# Autodesk Inventor assembly: AX-01 CoreXY
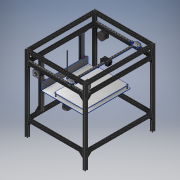
[picture p0: Inventor's stored thumbnail of the model, 180x180]
Saved by Autodesk Inventor 2017.3 (Build 213256000, 256)
## iProperties
Created: 2018-10-06
Part Number: AX-01 CoreXY
Document SubType Name: Assembly
Designer: Ax
Author: Ax
## Documents named in this file (36)
- C:\Users\Ax\Documents\Inventor\AX-01\AX-01 CoreXY.iam
- C:\Users\Ax\Documents\Inventor\Content Center Files\R2017\en-US\V-Slot 20 x 20\20-20-V-slot 20 mm x 20 mm-Aluminum 6061-470.ipt
- C:\Users\Ax\Documents\Inventor\Content Center Files\R2017\en-US\V-Slot 20 x 20\20-20-V-slot 20 mm x 20 mm-Aluminum 6061-550.ipt
- C:\Users\Ax\Documents\Inventor\Content Center Files\R2017\en-US\V-Slot 20 x 20\20-20-V-slot 20 mm x 20 mm-Aluminum 6061-400.ipt
- C:\Users\Ax\Documents\Inventor\Content Center Files\R2017\en-US\V-Slot 20 x 20\20-20-V-slot 20 mm x 20 mm-Aluminum 6061-340.ipt
- C:\Users\Ax\Documents\Inventor\AX-01\Bed Base.ipt
- C:\Users\Ax\Documents\Inventor\Drakon\Library\mgn12-sliding-block-linear-guide-1.snapshot.2\MGN12 Rail 300mm.ipt
- C:\Users\Ax\Documents\Inventor\Drakon\Library\mgn12-sliding-block-linear-guide-1.snapshot.2\MGN12H Block.iam
- C:\Users\Ax\Documents\Inventor\Drakon\Library\mgn12-sliding-block-linear-guide-1.snapshot.2\MGN12 Rail 300mm_MIR.ipt
- C:\Users\Ax\Documents\Inventor\Drakon\Library\mgn12-sliding-block-linear-guide-1.snapshot.2\MGN12H Block_MIR.iam
- C:\Users\Ax\Documents\Inventor\Drakon\Library\MGN9 Rail 400mm.ipt
- C:\Users\Ax\Documents\Inventor\Drakon\Library\MGN9C Block.ipt
- C:\Users\Ax\Documents\Inventor\Drakon\Library\MGN9 Rail 400mm_MIR.ipt
- C:\Users\Ax\Documents\Inventor\Drakon\Library\MGN9C Block_MIR.ipt
- C:\Users\Ax\Documents\Inventor\AX-01\Bed Plate.ipt
- C:\Users\Ax\Documents\Inventor\Drakon\Library\20mm Nylon Stand Off.ipt
- C:\Users\Ax\Documents\Inventor\AX-01\Internal Base Cladding.ipt
- C:\Users\Ax\Documents\Inventor\Drakon\Library\Nema 17 Motor.ipt
- C:\Users\Ax\Documents\Inventor\AX-01\300mmx8mm Lead Screw.ipt
- C:\Users\Ax\Documents\Inventor\Drakon\Library\Rigid_Coupler_5mm_8mm.iam
- C:\Users\Ax\Documents\Inventor\AX-01\TR8 Leadscrew Nut.ipt
- C:\Users\Ax\Documents\Inventor\AX-01\XY_Plate.ipt
- C:\Users\Ax\Documents\Inventor\AX-01\MGN-9 Rail 470mm.ipt
- C:\Users\Ax\Documents\Inventor\Content Center Files\R2017\en-US\ISO 4762(2)\ISO 4762 - M3 x 6ISO.ipt
- C:\Users\Ax\Documents\Inventor\AX-01\Back Cladding.ipt
- C:\Users\Ax\Documents\Inventor\AX-01\Side Cladding.ipt
- C:\Users\Ax\Documents\Inventor\AX-01\Front Cladding.ipt
- C:\Users\Ax\Documents\Inventor\AX-01\Top Cladding.ipt
- C:\Users\Ax\Documents\Inventor\AX-01\Corner Bracket.ipt
- C:\Users\Ax\Documents\Inventor\AX-01\Idler Pulley.iam
- C:\Users\Ax\Documents\Inventor\AX-01\XY_Carriage.ipt
- C:\Users\Ax\Documents\Inventor\AX-01\Idler Left.ipt
- C:\Users\Ax\Documents\Inventor\AX-01\XY_Tensioner.ipt
- C:\Users\Ax\Documents\Inventor\AX-01\XY_Metal_Slug.ipt
- C:\Users\Ax\Documents\Inventor\AX-01\M3 Conical Washer.ipt
- C:\Users\Ax\Documents\Inventor\AX-01\6mm XY Packer Block.ipt
## Components (114 placed, 35 different names)
1. Bed Base:1 — Mate:24, Mate:38, Mate:39, Flush:46, Mate:40, Mate:41, Mate:42, Mate:43, Mate:44, Mate:45, Mate:46, Mate:47, Mate:48, Mate:49, Mate:61, Mate:62, Mate:63
2. Bed Plate:1 — Mate:38, Mate:39, Flush:46
3. 20mm Nylon Stand Off:1 — Mate:46, Mate:47
4. 20mm Nylon Stand Off:2 — Mate:44, Mate:45
5. 20mm Nylon Stand Off:3 — Mate:40, Mate:41
6. 20mm Nylon Stand Off:4 — Mate:42, Mate:43
7. 300mmx8mm Lead Screw:1 — Mate:57, Mate:58
8. Rigid_Coupler_5mm_8mm:1 [sub-assembly] — Mate:57, Mate:58, Mate:59, Mate:60
9. TR8 Leadscrew Nut:1 — Mate:61, Mate:62, Mate:63
10. XY_Plate:1 — Mate:65, Mate:66, Mate:67, Mate:68, Mate:69, Mate:70, Insert:1, Insert:2, Insert:3, Insert:4, Mate:130, Mate:131, Rotational:4, Rotational:6, Rotational:7, Insert:6, Insert:7, Insert:8, Insert:9, Mate:172
11. Idler Pulley:2 [sub-assembly] — Mate:130, Mate:131
12. Idler Pulley:6 [sub-assembly] — Rotational:6
13. Idler Pulley:7 [sub-assembly] — Rotational:4
14. Idler Pulley:8 [sub-assembly] — Rotational:7
15. XY_Carriage:1 — Mate:151, Mate:152, Mate:153, Mate:154, Mate:155, Mate:156, Mate:157, Mate:158, Mate:159, Mate:160, Mate:161, Mate:162, Mate:163, Mate:164, Mate:165, Mate:166, Mate:167, Mate:168, Mate:169
16. Idler Left:1 — Mate:149, Mate:150, Flush:85
17. XY_Tensioner:1 — Mate:154, Mate:155, Mate:156
18. XY_Tensioner:2 — Mate:157, Mate:158, Mate:159
19. XY_Metal_Slug:1 — Mate:160, Mate:161
20. M3 Conical Washer:1 — Mate:163, Mate:169
21. M3 Conical Washer:2 — Mate:164, Mate:168
22. M3 Conical Washer:3 — Mate:162, Mate:167
23. M3 Conical Washer:4 — Mate:165, Mate:166
24. 6mm XY Packer Block:1 — Mate:170, Flush:86, Flush:87
25. 6mm XY Packer Block:2 — Mate:171, Flush:88, Flush:89, Mate:172
26. V-Slot 20 x 20 20-20-V-slot 20 mm x 20 mm-Aluminum 6061-340:2 — Flush:33, Flush:34, Mate:25, Mate:27, Mate:33, Flush:41, Flush:72, Mate:104, Flush:73, Mate:107, Flush:74, Mate:109
27. V-Slot 20 x 20 20-20-V-slot 20 mm x 20 mm-Aluminum 6061-340:1 — Mate:21, Mate:22, Flush:28, Flush:29, Mate:32, Flush:40, Mate:101, Flush:71, Mate:102, Flush:75, Mate:110, Flush:76, Mate:112
28. V-Slot 20 x 20 20-20-V-slot 20 mm x 20 mm-Aluminum 6061-550:1 — Mate:1, Flush:1, Flush:2, Mate:3, Flush:5, Flush:6, Mate:19, Flush:25, Flush:26, Flush:67, Mate:94, Flush:68, Mate:97, Flush:78, Mate:116, Flush:79, Mate:118
29. V-Slot 20 x 20 20-20-V-slot 20 mm x 20 mm-Aluminum 6061-550:2 — Mate:2, Flush:3, Flush:4, Mate:4, Flush:7, Mate:37, Mate:73, Mate:88, Flush:66, Mate:92, Flush:77, Mate:114, Flush:84, Mate:128
30. V-Slot 20 x 20 20-20-V-slot 20 mm x 20 mm-Aluminum 6061-470:1 — Mate:1, Flush:1, Flush:2, Mate:2, Flush:3, Flush:4, Mate:33, Flush:41, Mate:93, Mate:95, Flush:70, Mate:100, Mate:103, Mate:105, Mate:106
31. V-Slot 20 x 20 20-20-V-slot 20 mm x 20 mm-Aluminum 6061-470:2 — Mate:4, Flush:7, Mate:30, Mate:32, Flush:40, Mate:74, Mate:108, Mate:111, Mate:113, Mate:115, Mate:117
32. V-Slot 20 x 20 20-20-V-slot 20 mm x 20 mm-Aluminum 6061-470:3 — Mate:3, Flush:5, Flush:6, Mate:30
33. V-Slot 20 x 20 20-20-V-slot 20 mm x 20 mm-Aluminum 6061-550:3 — Flush:13, Mate:15, Mate:16, Mate:17, Flush:20, Flush:21, Flush:22, Flush:23, Flush:24, Mate:27, Flush:36, Mate:35, Flush:52, Flush:62, Mate:85, Flush:69, Mate:98, Flush:80, Mate:120, Flush:81, Mate:122, Mate:149
34. V-Slot 20 x 20 20-20-V-slot 20 mm x 20 mm-Aluminum 6061-550:4 — Mate:11, Flush:15, Flush:16, Mate:12, Flush:17, Mate:14, Flush:18, Flush:19, Mate:21, Flush:37, Flush:38, Flush:39, Mate:86, Flush:63, Flush:64, Mate:91, Flush:65, Flush:82, Mate:124, Flush:83, Mate:126
35. V-Slot 20 x 20 20-20-V-slot 20 mm x 20 mm-Aluminum 6061-470:4 — Flush:47, Mate:84, Mate:87
36. V-Slot 20 x 20 20-20-V-slot 20 mm x 20 mm-Aluminum 6061-470:5 — Mate:28, Mate:123, Mate:125, Mate:150, Flush:85
37. V-Slot 20 x 20 20-20-V-slot 20 mm x 20 mm-Aluminum 6061-470:6 — Flush:13, Mate:28, Mate:76
38. V-Slot 20 x 20 20-20-V-slot 20 mm x 20 mm-Aluminum 6061-400:1 — Mate:17, Flush:22, Flush:24, Mate:29, Mate:72, Flush:51, Mate:77
39. V-Slot 20 x 20 20-20-V-slot 20 mm x 20 mm-Aluminum 6061-400:2 — Mate:16, Flush:21, Mate:29, Mate:34, Flush:43, Mate:119, Mate:121
40. V-Slot 20 x 20 20-20-V-slot 20 mm x 20 mm-Aluminum 6061-400:3 — Mate:12, Flush:17, Mate:31, Mate:36, Flush:45, Mate:127, Mate:129
41. V-Slot 20 x 20 20-20-V-slot 20 mm x 20 mm-Aluminum 6061-400:4 — Mate:15, Flush:20, Flush:23, Mate:19, Flush:25, Flush:26, Mate:96, Mate:99
42. V-Slot 20 x 20 20-20-V-slot 20 mm x 20 mm-Aluminum 6061-400:5 — Mate:14, Flush:18, Flush:19, Mate:31, Flush:53
43. V-Slot 20 x 20 20-20-V-slot 20 mm x 20 mm-Aluminum 6061-400:6 — Mate:11, Flush:15, Flush:16, Mate:50, Flush:48, Mate:89, Mate:90
44. Internal Base Cladding:1 — Mate:50, Flush:47, Flush:48, Mate:51, Mate:52, Mate:53
45. Top Cladding:1 — Mate:77, Flush:60, Flush:61
46. Back Cladding:1 — Mate:74, Flush:56, Mate:75, Flush:57
47. Side Cladding:1 — Mate:73, Flush:53, Mate:75, Flush:57, Flush:58, Flush:59, Mate:78, Mate:79, Mate:80
48. Side Cladding:2 — Mate:72, Flush:51, Flush:52, Flush:56, Flush:60, Mate:81, Mate:82, Mate:83
49. Front Cladding:1 — Mate:76, Flush:58, Flush:59, Flush:61
50. MGN9C Block:2 — Slider:5, Mate:151, Mate:152, Mate:153
51. MGN-9 Rail 470mm:1 — Mate:68, Mate:69, Mate:70, Slider:5, Insert:5
52. MGN9C Block_MIR:1 — Slider:4, Mate:66, Mate:67, Mate:171, Flush:88, Flush:89
53. MGN9 Rail 400mm_MIR:1 — Slider:4, Mate:36, Mate:37, Flush:45
54. MGN9C Block:1 — Slider:3, Mate:65, Mate:170, Flush:86, Flush:87
55. MGN9 Rail 400mm:1 — Mate:34, Mate:35, Flush:43, Slider:3
56. MGN12H Block_MIR:1 [sub-assembly] — Mate:26, Slider:2, Mate:48
57. MGN12H Block:1 [sub-assembly] — Mate:23, Slider:1, Mate:24, Mate:49
58. MGN12 Rail 300mm:1 — Mate:22, Flush:28, Flush:29, Mate:23, Slider:1
59. MGN12 Rail 300mm_MIR:1 — Flush:33, Flush:34, Mate:25, Mate:26, Slider:2
60. Nema 17 Motor:2 — Mate:81, Mate:82, Mate:83
61. Nema 17 Motor:3 — Mate:78, Mate:79, Mate:80
62. Nema 17 Motor:1 — Mate:51, Mate:52, Mate:53, Mate:59, Mate:60
63. ISO 4762 M3 x 6:33 — Insert:8
64. ISO 4762 M3 x 6:34 — Insert:9
65. ISO 4762 M3 x 6:35 — Insert:6
66. ISO 4762 M3 x 6:36 — Insert:7
67. ISO 4762 M3 x 6:1 — Insert:3
68. ISO 4762 M3 x 6:2 — Insert:4
69. ISO 4762 M3 x 6:3 — Insert:1
70. ISO 4762 M3 x 6:4 — Insert:2
71. Corner Bracket:1 — Mate:84, Flush:62, Mate:85
72. Corner Bracket:2 — Flush:64, Mate:88, Mate:89
73. Corner Bracket:3 — Mate:86, Flush:63, Mate:87
74. Corner Bracket:4 — Flush:66, Mate:92, Mate:93
75. Corner Bracket:5 — Flush:67, Mate:94, Mate:95
76. Corner Bracket:6 — Mate:90, Mate:91, Flush:65
77. Corner Bracket:7 — Flush:83, Mate:126, Mate:127
78. Corner Bracket:8 — Flush:69, Mate:98, Mate:99
79. Corner Bracket:9 — Flush:68, Mate:96, Mate:97
80. Corner Bracket:10 — Flush:75, Mate:110, Mate:111
81. Corner Bracket:11 — Flush:70, Mate:100, Mate:101
82. Corner Bracket:12 — Flush:76, Mate:112, Mate:113
83. Corner Bracket:13 — Flush:78, Mate:116, Mate:117
84. Corner Bracket:14 — Flush:74, Mate:108, Mate:109
85. Corner Bracket:15 — Flush:72, Mate:104, Mate:105
86. Corner Bracket:16 — Flush:71, Mate:102, Mate:103
87. Corner Bracket:17 — Flush:73, Mate:106, Mate:107
88. Corner Bracket:18 — Flush:77, Mate:114, Mate:115
89. Corner Bracket:19 — Flush:82, Mate:124, Mate:125
90. Corner Bracket:20 — Flush:81, Mate:122, Mate:123
91. Corner Bracket:21 — Flush:79, Mate:118, Mate:119
92. Corner Bracket:22 — Flush:80, Mate:120, Mate:121
93. Corner Bracket:23 — Flush:84, Mate:128, Mate:129
94. ISO 4762 M3 x 6:12 — Insert:5
95. ISO 4762 M3 x 6:13
96. ISO 4762 M3 x 6:14
97. ISO 4762 M3 x 6:15
98. ISO 4762 M3 x 6:16
99. ISO 4762 M3 x 6:17
100. ISO 4762 M3 x 6:18
101. ISO 4762 M3 x 6:19
102. ISO 4762 M3 x 6:20
103. ISO 4762 M3 x 6:21
104. ISO 4762 M3 x 6:22
105. ISO 4762 M3 x 6:23
106. ISO 4762 M3 x 6:24
107. ISO 4762 M3 x 6:25
108. ISO 4762 M3 x 6:26
109. ISO 4762 M3 x 6:27
110. ISO 4762 M3 x 6:28
111. ISO 4762 M3 x 6:29
112. ISO 4762 M3 x 6:30
113. ISO 4762 M3 x 6:31
114. ISO 4762 M3 x 6:32
## Component patterns: (21 elements, first: ISO 4762 M3 x 6:12)
## Relationships (241: Mate 145, Flush 79, Insert 9, TranslationJoint 5, RevoluteJoint 3)
- Mate:1: V-Slot 20 x 20 20-20-V-slot 20 mm x 20 mm-Aluminum 6061-550:1 ↔ V-Slot 20 x 20 20-20-V-slot 20 mm x 20 mm-Aluminum 6061-470:1
- Flush:1 (100 mm): V-Slot 20 x 20 20-20-V-slot 20 mm x 20 mm-Aluminum 6061-550:1 ↔ V-Slot 20 x 20 20-20-V-slot 20 mm x 20 mm-Aluminum 6061-470:1
- Flush:2: V-Slot 20 x 20 20-20-V-slot 20 mm x 20 mm-Aluminum 6061-550:1 ↔ V-Slot 20 x 20 20-20-V-slot 20 mm x 20 mm-Aluminum 6061-470:1
- Mate:2: V-Slot 20 x 20 20-20-V-slot 20 mm x 20 mm-Aluminum 6061-550:2 ↔ V-Slot 20 x 20 20-20-V-slot 20 mm x 20 mm-Aluminum 6061-470:1
- Flush:3 (-100 mm): V-Slot 20 x 20 20-20-V-slot 20 mm x 20 mm-Aluminum 6061-550:2 ↔ V-Slot 20 x 20 20-20-V-slot 20 mm x 20 mm-Aluminum 6061-470:1
- Flush:4: V-Slot 20 x 20 20-20-V-slot 20 mm x 20 mm-Aluminum 6061-550:2 ↔ V-Slot 20 x 20 20-20-V-slot 20 mm x 20 mm-Aluminum 6061-470:1
- Mate:3: V-Slot 20 x 20 20-20-V-slot 20 mm x 20 mm-Aluminum 6061-550:1 ↔ V-Slot 20 x 20 20-20-V-slot 20 mm x 20 mm-Aluminum 6061-470:3
- Flush:5: V-Slot 20 x 20 20-20-V-slot 20 mm x 20 mm-Aluminum 6061-550:1 ↔ V-Slot 20 x 20 20-20-V-slot 20 mm x 20 mm-Aluminum 6061-470:3
- Flush:6: V-Slot 20 x 20 20-20-V-slot 20 mm x 20 mm-Aluminum 6061-550:1 ↔ V-Slot 20 x 20 20-20-V-slot 20 mm x 20 mm-Aluminum 6061-470:3
- Mate:4: V-Slot 20 x 20 20-20-V-slot 20 mm x 20 mm-Aluminum 6061-550:2 ↔ V-Slot 20 x 20 20-20-V-slot 20 mm x 20 mm-Aluminum 6061-470:2
- Flush:7: V-Slot 20 x 20 20-20-V-slot 20 mm x 20 mm-Aluminum 6061-550:2 ↔ V-Slot 20 x 20 20-20-V-slot 20 mm x 20 mm-Aluminum 6061-470:2
- [Mate]: V-Slot 20 x 20 20-20-V-slot 20 mm x 20 mm-Aluminum 6061-550:3 ↔ V-Slot 20 x 20 20-20-V-slot 20 mm x 20 mm-Aluminum 6061-470:4
- [Flush] (100 mm): V-Slot 20 x 20 20-20-V-slot 20 mm x 20 mm-Aluminum 6061-550:3 ↔ V-Slot 20 x 20 20-20-V-slot 20 mm x 20 mm-Aluminum 6061-470:4
- [Flush]: V-Slot 20 x 20 20-20-V-slot 20 mm x 20 mm-Aluminum 6061-550:3 ↔ V-Slot 20 x 20 20-20-V-slot 20 mm x 20 mm-Aluminum 6061-470:4
- [Mate]: V-Slot 20 x 20 20-20-V-slot 20 mm x 20 mm-Aluminum 6061-550:4 ↔ V-Slot 20 x 20 20-20-V-slot 20 mm x 20 mm-Aluminum 6061-470:4
- [Flush] (-100 mm): V-Slot 20 x 20 20-20-V-slot 20 mm x 20 mm-Aluminum 6061-550:4 ↔ V-Slot 20 x 20 20-20-V-slot 20 mm x 20 mm-Aluminum 6061-470:4
- [Flush]: V-Slot 20 x 20 20-20-V-slot 20 mm x 20 mm-Aluminum 6061-550:4 ↔ V-Slot 20 x 20 20-20-V-slot 20 mm x 20 mm-Aluminum 6061-470:4
- [Mate]: V-Slot 20 x 20 20-20-V-slot 20 mm x 20 mm-Aluminum 6061-550:3 ↔ V-Slot 20 x 20 20-20-V-slot 20 mm x 20 mm-Aluminum 6061-470:6
- [Flush]: V-Slot 20 x 20 20-20-V-slot 20 mm x 20 mm-Aluminum 6061-550:3 ↔ V-Slot 20 x 20 20-20-V-slot 20 mm x 20 mm-Aluminum 6061-470:6
- Flush:13: V-Slot 20 x 20 20-20-V-slot 20 mm x 20 mm-Aluminum 6061-550:3 ↔ V-Slot 20 x 20 20-20-V-slot 20 mm x 20 mm-Aluminum 6061-470:6
- [Mate]: V-Slot 20 x 20 20-20-V-slot 20 mm x 20 mm-Aluminum 6061-550:4 ↔ V-Slot 20 x 20 20-20-V-slot 20 mm x 20 mm-Aluminum 6061-470:5
- [Flush]: V-Slot 20 x 20 20-20-V-slot 20 mm x 20 mm-Aluminum 6061-550:4 ↔ V-Slot 20 x 20 20-20-V-slot 20 mm x 20 mm-Aluminum 6061-470:5
- Mate:11: V-Slot 20 x 20 20-20-V-slot 20 mm x 20 mm-Aluminum 6061-550:4 ↔ V-Slot 20 x 20 20-20-V-slot 20 mm x 20 mm-Aluminum 6061-400:6
- Flush:15 (100 mm): V-Slot 20 x 20 20-20-V-slot 20 mm x 20 mm-Aluminum 6061-550:4 ↔ V-Slot 20 x 20 20-20-V-slot 20 mm x 20 mm-Aluminum 6061-400:6
- Flush:16: V-Slot 20 x 20 20-20-V-slot 20 mm x 20 mm-Aluminum 6061-550:4 ↔ V-Slot 20 x 20 20-20-V-slot 20 mm x 20 mm-Aluminum 6061-400:6
- Mate:12: V-Slot 20 x 20 20-20-V-slot 20 mm x 20 mm-Aluminum 6061-550:4 ↔ V-Slot 20 x 20 20-20-V-slot 20 mm x 20 mm-Aluminum 6061-400:3
- Flush:17: V-Slot 20 x 20 20-20-V-slot 20 mm x 20 mm-Aluminum 6061-550:4 ↔ V-Slot 20 x 20 20-20-V-slot 20 mm x 20 mm-Aluminum 6061-400:3
- Mate:14: V-Slot 20 x 20 20-20-V-slot 20 mm x 20 mm-Aluminum 6061-550:4 ↔ V-Slot 20 x 20 20-20-V-slot 20 mm x 20 mm-Aluminum 6061-400:5
- Flush:18: V-Slot 20 x 20 20-20-V-slot 20 mm x 20 mm-Aluminum 6061-550:4 ↔ V-Slot 20 x 20 20-20-V-slot 20 mm x 20 mm-Aluminum 6061-400:5
- Flush:19: V-Slot 20 x 20 20-20-V-slot 20 mm x 20 mm-Aluminum 6061-550:4 ↔ V-Slot 20 x 20 20-20-V-slot 20 mm x 20 mm-Aluminum 6061-400:5
- Mate:15: V-Slot 20 x 20 20-20-V-slot 20 mm x 20 mm-Aluminum 6061-550:3 ↔ V-Slot 20 x 20 20-20-V-slot 20 mm x 20 mm-Aluminum 6061-400:4
- Mate:16: V-Slot 20 x 20 20-20-V-slot 20 mm x 20 mm-Aluminum 6061-550:3 ↔ V-Slot 20 x 20 20-20-V-slot 20 mm x 20 mm-Aluminum 6061-400:2
- Mate:17: V-Slot 20 x 20 20-20-V-slot 20 mm x 20 mm-Aluminum 6061-550:3 ↔ V-Slot 20 x 20 20-20-V-slot 20 mm x 20 mm-Aluminum 6061-400:1
- Flush:20: V-Slot 20 x 20 20-20-V-slot 20 mm x 20 mm-Aluminum 6061-550:3 ↔ V-Slot 20 x 20 20-20-V-slot 20 mm x 20 mm-Aluminum 6061-400:4
- Flush:21: V-Slot 20 x 20 20-20-V-slot 20 mm x 20 mm-Aluminum 6061-550:3 ↔ V-Slot 20 x 20 20-20-V-slot 20 mm x 20 mm-Aluminum 6061-400:2
- Flush:22: V-Slot 20 x 20 20-20-V-slot 20 mm x 20 mm-Aluminum 6061-550:3 ↔ V-Slot 20 x 20 20-20-V-slot 20 mm x 20 mm-Aluminum 6061-400:1
- Flush:23 (100 mm): V-Slot 20 x 20 20-20-V-slot 20 mm x 20 mm-Aluminum 6061-550:3 ↔ V-Slot 20 x 20 20-20-V-slot 20 mm x 20 mm-Aluminum 6061-400:4
- Flush:24: V-Slot 20 x 20 20-20-V-slot 20 mm x 20 mm-Aluminum 6061-550:3 ↔ V-Slot 20 x 20 20-20-V-slot 20 mm x 20 mm-Aluminum 6061-400:1
- Mate:19: V-Slot 20 x 20 20-20-V-slot 20 mm x 20 mm-Aluminum 6061-550:1 ↔ V-Slot 20 x 20 20-20-V-slot 20 mm x 20 mm-Aluminum 6061-400:4
- Flush:25 (100 mm): V-Slot 20 x 20 20-20-V-slot 20 mm x 20 mm-Aluminum 6061-550:1 ↔ V-Slot 20 x 20 20-20-V-slot 20 mm x 20 mm-Aluminum 6061-400:4
- Flush:26: V-Slot 20 x 20 20-20-V-slot 20 mm x 20 mm-Aluminum 6061-550:1 ↔ V-Slot 20 x 20 20-20-V-slot 20 mm x 20 mm-Aluminum 6061-400:4
- Mate:21 (78.5 mm): V-Slot 20 x 20 20-20-V-slot 20 mm x 20 mm-Aluminum 6061-340:1 ↔ V-Slot 20 x 20 20-20-V-slot 20 mm x 20 mm-Aluminum 6061-550:4
- Mate:22: V-Slot 20 x 20 20-20-V-slot 20 mm x 20 mm-Aluminum 6061-340:1 ↔ MGN12 Rail 300mm:1
- Flush:28: V-Slot 20 x 20 20-20-V-slot 20 mm x 20 mm-Aluminum 6061-340:1 ↔ MGN12 Rail 300mm:1
- Flush:29 (4 mm): V-Slot 20 x 20 20-20-V-slot 20 mm x 20 mm-Aluminum 6061-340:1 ↔ MGN12 Rail 300mm:1
- Mate:23: MGN12H Block:1 ↔ MGN12 Rail 300mm:1
- Slider:1 [TranslationJoint]: MGN12H Block:1 ↔ MGN12 Rail 300mm:1
- Mate:24: Bed Base:1 ↔ MGN12H Block:1
- Flush:33 (4 mm): V-Slot 20 x 20 20-20-V-slot 20 mm x 20 mm-Aluminum 6061-340:2 ↔ MGN12 Rail 300mm_MIR:1
- Flush:34: V-Slot 20 x 20 20-20-V-slot 20 mm x 20 mm-Aluminum 6061-340:2 ↔ MGN12 Rail 300mm_MIR:1
- Mate:25: V-Slot 20 x 20 20-20-V-slot 20 mm x 20 mm-Aluminum 6061-340:2 ↔ MGN12 Rail 300mm_MIR:1
- Mate:26: MGN12H Block_MIR:1 ↔ MGN12 Rail 300mm_MIR:1
- Slider:2 [TranslationJoint]: MGN12H Block_MIR:1 ↔ MGN12 Rail 300mm_MIR:1
- Mate:27 (78.5 mm): V-Slot 20 x 20 20-20-V-slot 20 mm x 20 mm-Aluminum 6061-340:2 ↔ V-Slot 20 x 20 20-20-V-slot 20 mm x 20 mm-Aluminum 6061-550:3
- Flush:36: V-Slot 20 x 20 20-20-V-slot 20 mm x 20 mm-Aluminum 6061-550:3
- Mate:28 (50 mm): V-Slot 20 x 20 20-20-V-slot 20 mm x 20 mm-Aluminum 6061-470:5 ↔ V-Slot 20 x 20 20-20-V-slot 20 mm x 20 mm-Aluminum 6061-470:6
- Mate:29 (50 mm): V-Slot 20 x 20 20-20-V-slot 20 mm x 20 mm-Aluminum 6061-400:1 ↔ V-Slot 20 x 20 20-20-V-slot 20 mm x 20 mm-Aluminum 6061-400:2
- Mate:30 (50 mm): V-Slot 20 x 20 20-20-V-slot 20 mm x 20 mm-Aluminum 6061-470:2 ↔ V-Slot 20 x 20 20-20-V-slot 20 mm x 20 mm-Aluminum 6061-470:3
- Mate:31 (50 mm): V-Slot 20 x 20 20-20-V-slot 20 mm x 20 mm-Aluminum 6061-400:3 ↔ V-Slot 20 x 20 20-20-V-slot 20 mm x 20 mm-Aluminum 6061-400:5
- Flush:37: V-Slot 20 x 20 20-20-V-slot 20 mm x 20 mm-Aluminum 6061-550:4
- Flush:38: V-Slot 20 x 20 20-20-V-slot 20 mm x 20 mm-Aluminum 6061-550:4
- Flush:39: V-Slot 20 x 20 20-20-V-slot 20 mm x 20 mm-Aluminum 6061-550:4
- Mate:32: V-Slot 20 x 20 20-20-V-slot 20 mm x 20 mm-Aluminum 6061-340:1 ↔ V-Slot 20 x 20 20-20-V-slot 20 mm x 20 mm-Aluminum 6061-470:2
- Flush:40: V-Slot 20 x 20 20-20-V-slot 20 mm x 20 mm-Aluminum 6061-340:1 ↔ V-Slot 20 x 20 20-20-V-slot 20 mm x 20 mm-Aluminum 6061-470:2
- Mate:33: V-Slot 20 x 20 20-20-V-slot 20 mm x 20 mm-Aluminum 6061-340:2 ↔ V-Slot 20 x 20 20-20-V-slot 20 mm x 20 mm-Aluminum 6061-470:1
- Flush:41: V-Slot 20 x 20 20-20-V-slot 20 mm x 20 mm-Aluminum 6061-340:2 ↔ V-Slot 20 x 20 20-20-V-slot 20 mm x 20 mm-Aluminum 6061-470:1
- Mate:34: V-Slot 20 x 20 20-20-V-slot 20 mm x 20 mm-Aluminum 6061-400:2 ↔ MGN9 Rail 400mm:1
- Mate:35: V-Slot 20 x 20 20-20-V-slot 20 mm x 20 mm-Aluminum 6061-550:3 ↔ MGN9 Rail 400mm:1
- Flush:43 (5.5 mm): V-Slot 20 x 20 20-20-V-slot 20 mm x 20 mm-Aluminum 6061-400:2 ↔ MGN9 Rail 400mm:1
- Slider:3 [TranslationJoint]: MGN9C Block:1 ↔ MGN9 Rail 400mm:1
- Flush:44 (-255 mm)
- Slider:4 [TranslationJoint]: MGN9C Block_MIR:1 ↔ MGN9 Rail 400mm_MIR:1
- Mate:36: V-Slot 20 x 20 20-20-V-slot 20 mm x 20 mm-Aluminum 6061-400:3 ↔ MGN9 Rail 400mm_MIR:1
- Mate:37: V-Slot 20 x 20 20-20-V-slot 20 mm x 20 mm-Aluminum 6061-550:2 ↔ MGN9 Rail 400mm_MIR:1
- Flush:45 (5.5 mm): V-Slot 20 x 20 20-20-V-slot 20 mm x 20 mm-Aluminum 6061-400:3 ↔ MGN9 Rail 400mm_MIR:1
- Mate:38 (20 mm): Bed Base:1 ↔ Bed Plate:1
- Mate:39 (84 mm): Bed Base:1 ↔ Bed Plate:1
- Flush:46 (10 mm): Bed Base:1 ↔ Bed Plate:1
- Mate:40: Bed Base:1 ↔ 20mm Nylon Stand Off:3
- Mate:41: Bed Base:1 ↔ 20mm Nylon Stand Off:3
- Mate:42: Bed Base:1 ↔ 20mm Nylon Stand Off:4
- Mate:43: Bed Base:1 ↔ 20mm Nylon Stand Off:4
- Mate:44: Bed Base:1 ↔ 20mm Nylon Stand Off:2
- Mate:45: Bed Base:1 ↔ 20mm Nylon Stand Off:2
- Mate:46: Bed Base:1 ↔ 20mm Nylon Stand Off:1
- Mate:47: Bed Base:1 ↔ 20mm Nylon Stand Off:1
- Mate:48: Bed Base:1 ↔ MGN12H Block_MIR:1
- Mate:49: Bed Base:1 ↔ MGN12H Block:1
- Mate:50: V-Slot 20 x 20 20-20-V-slot 20 mm x 20 mm-Aluminum 6061-400:6 ↔ Internal Base Cladding:1
- Flush:47: V-Slot 20 x 20 20-20-V-slot 20 mm x 20 mm-Aluminum 6061-470:4 ↔ Internal Base Cladding:1
- Flush:48: V-Slot 20 x 20 20-20-V-slot 20 mm x 20 mm-Aluminum 6061-400:6 ↔ Internal Base Cladding:1
- Mate:51: Internal Base Cladding:1 ↔ Nema 17 Motor:1
- Mate:52: Internal Base Cladding:1 ↔ Nema 17 Motor:1
- Mate:53: Internal Base Cladding:1 ↔ Nema 17 Motor:1
- Mate:57: 300mmx8mm Lead Screw:1 ↔ Rigid_Coupler_5mm_8mm:1
- Mate:58: 300mmx8mm Lead Screw:1 ↔ Rigid_Coupler_5mm_8mm:1
- Mate:59 (7 mm): Rigid_Coupler_5mm_8mm:1 ↔ Nema 17 Motor:1
- Mate:60: Rigid_Coupler_5mm_8mm:1 ↔ Nema 17 Motor:1
- Mate:61: Bed Base:1 ↔ TR8 Leadscrew Nut:1
- Mate:62: Bed Base:1 ↔ TR8 Leadscrew Nut:1
- Mate:63: Bed Base:1 ↔ TR8 Leadscrew Nut:1
- Mate:65: XY_Plate:1 ↔ MGN9C Block:1
- Mate:66: XY_Plate:1 ↔ MGN9C Block_MIR:1
- Mate:67: XY_Plate:1 ↔ MGN9C Block_MIR:1
- Mate:68: XY_Plate:1 ↔ MGN-9 Rail 470mm:1
- Mate:69: XY_Plate:1 ↔ MGN-9 Rail 470mm:1
- Mate:70: XY_Plate:1 ↔ MGN-9 Rail 470mm:1
- Slider:5 [TranslationJoint]: MGN9C Block:2 ↔ MGN-9 Rail 470mm:1
- Insert:1: XY_Plate:1 ↔ ISO 4762 M3 x 6:3
- Insert:2: XY_Plate:1 ↔ ISO 4762 M3 x 6:4
- Insert:3: XY_Plate:1 ↔ ISO 4762 M3 x 6:1
- Insert:4: XY_Plate:1 ↔ ISO 4762 M3 x 6:2
- Mate:72: V-Slot 20 x 20 20-20-V-slot 20 mm x 20 mm-Aluminum 6061-400:1 ↔ Side Cladding:2
- Flush:51: V-Slot 20 x 20 20-20-V-slot 20 mm x 20 mm-Aluminum 6061-400:1 ↔ Side Cladding:2
- Flush:52: V-Slot 20 x 20 20-20-V-slot 20 mm x 20 mm-Aluminum 6061-550:3 ↔ Side Cladding:2
- Mate:73: V-Slot 20 x 20 20-20-V-slot 20 mm x 20 mm-Aluminum 6061-550:2 ↔ Side Cladding:1
- Flush:53: V-Slot 20 x 20 20-20-V-slot 20 mm x 20 mm-Aluminum 6061-400:5 ↔ Side Cladding:1
- Mate:74: V-Slot 20 x 20 20-20-V-slot 20 mm x 20 mm-Aluminum 6061-470:2 ↔ Back Cladding:1
- Flush:56: Back Cladding:1 ↔ Side Cladding:2
- Mate:75: Back Cladding:1 ↔ Side Cladding:1
- Flush:57: Back Cladding:1 ↔ Side Cladding:1
- Mate:76: V-Slot 20 x 20 20-20-V-slot 20 mm x 20 mm-Aluminum 6061-470:6 ↔ Front Cladding:1
- Flush:58: Side Cladding:1 ↔ Front Cladding:1
- Flush:59: Side Cladding:1 ↔ Front Cladding:1
- Mate:77: V-Slot 20 x 20 20-20-V-slot 20 mm x 20 mm-Aluminum 6061-400:1 ↔ Top Cladding:1
- Flush:60: Top Cladding:1 ↔ Side Cladding:2
- Flush:61: Top Cladding:1 ↔ Front Cladding:1
- Mate:78: Side Cladding:1 ↔ Nema 17 Motor:3
- Mate:79: Side Cladding:1 ↔ Nema 17 Motor:3
- Mate:80: Side Cladding:1 ↔ Nema 17 Motor:3
- Mate:81: Side Cladding:2 ↔ Nema 17 Motor:2
- Mate:82: Side Cladding:2 ↔ Nema 17 Motor:2
- Mate:83: Side Cladding:2 ↔ Nema 17 Motor:2
- Mate:84: V-Slot 20 x 20 20-20-V-slot 20 mm x 20 mm-Aluminum 6061-470:4 ↔ Corner Bracket:1
- Flush:62: V-Slot 20 x 20 20-20-V-slot 20 mm x 20 mm-Aluminum 6061-550:3 ↔ Corner Bracket:1
- Mate:85: V-Slot 20 x 20 20-20-V-slot 20 mm x 20 mm-Aluminum 6061-550:3 ↔ Corner Bracket:1
- Mate:86: V-Slot 20 x 20 20-20-V-slot 20 mm x 20 mm-Aluminum 6061-550:4 ↔ Corner Bracket:3
- Flush:63: V-Slot 20 x 20 20-20-V-slot 20 mm x 20 mm-Aluminum 6061-550:4 ↔ Corner Bracket:3
- Mate:87: V-Slot 20 x 20 20-20-V-slot 20 mm x 20 mm-Aluminum 6061-470:4 ↔ Corner Bracket:3
- Flush:64: V-Slot 20 x 20 20-20-V-slot 20 mm x 20 mm-Aluminum 6061-550:4 ↔ Corner Bracket:2
- Mate:88: V-Slot 20 x 20 20-20-V-slot 20 mm x 20 mm-Aluminum 6061-550:2 ↔ Corner Bracket:2
- Mate:89: V-Slot 20 x 20 20-20-V-slot 20 mm x 20 mm-Aluminum 6061-400:6 ↔ Corner Bracket:2
- Mate:90: V-Slot 20 x 20 20-20-V-slot 20 mm x 20 mm-Aluminum 6061-400:6 ↔ Corner Bracket:6
- Mate:91: V-Slot 20 x 20 20-20-V-slot 20 mm x 20 mm-Aluminum 6061-550:4 ↔ Corner Bracket:6
- Flush:65: V-Slot 20 x 20 20-20-V-slot 20 mm x 20 mm-Aluminum 6061-550:4 ↔ Corner Bracket:6
- Flush:66: V-Slot 20 x 20 20-20-V-slot 20 mm x 20 mm-Aluminum 6061-550:2 ↔ Corner Bracket:4
- Mate:92: V-Slot 20 x 20 20-20-V-slot 20 mm x 20 mm-Aluminum 6061-550:2 ↔ Corner Bracket:4
- Mate:93: V-Slot 20 x 20 20-20-V-slot 20 mm x 20 mm-Aluminum 6061-470:1 ↔ Corner Bracket:4
- Flush:67: V-Slot 20 x 20 20-20-V-slot 20 mm x 20 mm-Aluminum 6061-550:1 ↔ Corner Bracket:5
- Mate:94: V-Slot 20 x 20 20-20-V-slot 20 mm x 20 mm-Aluminum 6061-550:1 ↔ Corner Bracket:5
- Mate:95: V-Slot 20 x 20 20-20-V-slot 20 mm x 20 mm-Aluminum 6061-470:1 ↔ Corner Bracket:5
- Flush:68: V-Slot 20 x 20 20-20-V-slot 20 mm x 20 mm-Aluminum 6061-550:1 ↔ Corner Bracket:9
- Mate:96: V-Slot 20 x 20 20-20-V-slot 20 mm x 20 mm-Aluminum 6061-400:4 ↔ Corner Bracket:9
- Mate:97: V-Slot 20 x 20 20-20-V-slot 20 mm x 20 mm-Aluminum 6061-550:1 ↔ Corner Bracket:9
- Flush:69: V-Slot 20 x 20 20-20-V-slot 20 mm x 20 mm-Aluminum 6061-550:3 ↔ Corner Bracket:8
- Mate:98: V-Slot 20 x 20 20-20-V-slot 20 mm x 20 mm-Aluminum 6061-550:3 ↔ Corner Bracket:8
- Mate:99: V-Slot 20 x 20 20-20-V-slot 20 mm x 20 mm-Aluminum 6061-400:4 ↔ Corner Bracket:8
- Flush:70: V-Slot 20 x 20 20-20-V-slot 20 mm x 20 mm-Aluminum 6061-470:1 ↔ Corner Bracket:11
- Mate:100: V-Slot 20 x 20 20-20-V-slot 20 mm x 20 mm-Aluminum 6061-470:1 ↔ Corner Bracket:11
- Mate:101: V-Slot 20 x 20 20-20-V-slot 20 mm x 20 mm-Aluminum 6061-340:1 ↔ Corner Bracket:11
- Flush:71: V-Slot 20 x 20 20-20-V-slot 20 mm x 20 mm-Aluminum 6061-340:1 ↔ Corner Bracket:16
- Mate:102: V-Slot 20 x 20 20-20-V-slot 20 mm x 20 mm-Aluminum 6061-340:1 ↔ Corner Bracket:16
- Mate:103: V-Slot 20 x 20 20-20-V-slot 20 mm x 20 mm-Aluminum 6061-470:1 ↔ Corner Bracket:16
- Flush:72: V-Slot 20 x 20 20-20-V-slot 20 mm x 20 mm-Aluminum 6061-340:2 ↔ Corner Bracket:15
- Mate:104: V-Slot 20 x 20 20-20-V-slot 20 mm x 20 mm-Aluminum 6061-340:2 ↔ Corner Bracket:15
- Mate:105: V-Slot 20 x 20 20-20-V-slot 20 mm x 20 mm-Aluminum 6061-470:1 ↔ Corner Bracket:15
- Flush:73: V-Slot 20 x 20 20-20-V-slot 20 mm x 20 mm-Aluminum 6061-340:2 ↔ Corner Bracket:17
- Mate:106: V-Slot 20 x 20 20-20-V-slot 20 mm x 20 mm-Aluminum 6061-470:1 ↔ Corner Bracket:17
- Mate:107: V-Slot 20 x 20 20-20-V-slot 20 mm x 20 mm-Aluminum 6061-340:2 ↔ Corner Bracket:17
- Flush:74: V-Slot 20 x 20 20-20-V-slot 20 mm x 20 mm-Aluminum 6061-340:2 ↔ Corner Bracket:14
- Mate:108: V-Slot 20 x 20 20-20-V-slot 20 mm x 20 mm-Aluminum 6061-470:2 ↔ Corner Bracket:14
- Mate:109: V-Slot 20 x 20 20-20-V-slot 20 mm x 20 mm-Aluminum 6061-340:2 ↔ Corner Bracket:14
- Flush:75: V-Slot 20 x 20 20-20-V-slot 20 mm x 20 mm-Aluminum 6061-340:1 ↔ Corner Bracket:10
- Mate:110: V-Slot 20 x 20 20-20-V-slot 20 mm x 20 mm-Aluminum 6061-340:1 ↔ Corner Bracket:10
- Mate:111: V-Slot 20 x 20 20-20-V-slot 20 mm x 20 mm-Aluminum 6061-470:2 ↔ Corner Bracket:10
- Flush:76: V-Slot 20 x 20 20-20-V-slot 20 mm x 20 mm-Aluminum 6061-340:1 ↔ Corner Bracket:12
- Mate:112: V-Slot 20 x 20 20-20-V-slot 20 mm x 20 mm-Aluminum 6061-340:1 ↔ Corner Bracket:12
- Mate:113: V-Slot 20 x 20 20-20-V-slot 20 mm x 20 mm-Aluminum 6061-470:2 ↔ Corner Bracket:12
- Flush:77: V-Slot 20 x 20 20-20-V-slot 20 mm x 20 mm-Aluminum 6061-550:2 ↔ Corner Bracket:18
- Mate:114: V-Slot 20 x 20 20-20-V-slot 20 mm x 20 mm-Aluminum 6061-550:2 ↔ Corner Bracket:18
- Mate:115: V-Slot 20 x 20 20-20-V-slot 20 mm x 20 mm-Aluminum 6061-470:2 ↔ Corner Bracket:18
- Flush:78: V-Slot 20 x 20 20-20-V-slot 20 mm x 20 mm-Aluminum 6061-550:1 ↔ Corner Bracket:13
- Mate:116: V-Slot 20 x 20 20-20-V-slot 20 mm x 20 mm-Aluminum 6061-550:1 ↔ Corner Bracket:13
- Mate:117: V-Slot 20 x 20 20-20-V-slot 20 mm x 20 mm-Aluminum 6061-470:2 ↔ Corner Bracket:13
- Flush:79: V-Slot 20 x 20 20-20-V-slot 20 mm x 20 mm-Aluminum 6061-550:1 ↔ Corner Bracket:21
- Mate:118: V-Slot 20 x 20 20-20-V-slot 20 mm x 20 mm-Aluminum 6061-550:1 ↔ Corner Bracket:21
- Mate:119: V-Slot 20 x 20 20-20-V-slot 20 mm x 20 mm-Aluminum 6061-400:2 ↔ Corner Bracket:21
- Flush:80: V-Slot 20 x 20 20-20-V-slot 20 mm x 20 mm-Aluminum 6061-550:3 ↔ Corner Bracket:22
- Mate:120: V-Slot 20 x 20 20-20-V-slot 20 mm x 20 mm-Aluminum 6061-550:3 ↔ Corner Bracket:22
- Mate:121: V-Slot 20 x 20 20-20-V-slot 20 mm x 20 mm-Aluminum 6061-400:2 ↔ Corner Bracket:22
- Flush:81: V-Slot 20 x 20 20-20-V-slot 20 mm x 20 mm-Aluminum 6061-550:3 ↔ Corner Bracket:20
- Mate:122: V-Slot 20 x 20 20-20-V-slot 20 mm x 20 mm-Aluminum 6061-550:3 ↔ Corner Bracket:20
- Mate:123: V-Slot 20 x 20 20-20-V-slot 20 mm x 20 mm-Aluminum 6061-470:5 ↔ Corner Bracket:20
- Flush:82: V-Slot 20 x 20 20-20-V-slot 20 mm x 20 mm-Aluminum 6061-550:4 ↔ Corner Bracket:19
- Mate:124: V-Slot 20 x 20 20-20-V-slot 20 mm x 20 mm-Aluminum 6061-550:4 ↔ Corner Bracket:19
- Mate:125: V-Slot 20 x 20 20-20-V-slot 20 mm x 20 mm-Aluminum 6061-470:5 ↔ Corner Bracket:19
- Flush:83: V-Slot 20 x 20 20-20-V-slot 20 mm x 20 mm-Aluminum 6061-550:4 ↔ Corner Bracket:7
- Mate:126: V-Slot 20 x 20 20-20-V-slot 20 mm x 20 mm-Aluminum 6061-550:4 ↔ Corner Bracket:7
- Mate:127: V-Slot 20 x 20 20-20-V-slot 20 mm x 20 mm-Aluminum 6061-400:3 ↔ Corner Bracket:7
- Flush:84: V-Slot 20 x 20 20-20-V-slot 20 mm x 20 mm-Aluminum 6061-550:2 ↔ Corner Bracket:23
- Mate:128: V-Slot 20 x 20 20-20-V-slot 20 mm x 20 mm-Aluminum 6061-550:2 ↔ Corner Bracket:23
- Mate:129: V-Slot 20 x 20 20-20-V-slot 20 mm x 20 mm-Aluminum 6061-400:3 ↔ Corner Bracket:23
- Mate:130: XY_Plate:1 ↔ Idler Pulley:2
- Mate:131: XY_Plate:1 ↔ Idler Pulley:2
- Rotational:4 [RevoluteJoint]: XY_Plate:1 ↔ Idler Pulley:7
- Rotational:6 [RevoluteJoint]: XY_Plate:1 ↔ Idler Pulley:6
- Rotational:7 [RevoluteJoint]: XY_Plate:1 ↔ Idler Pulley:8
- Insert:5: MGN-9 Rail 470mm:1 ↔ ISO 4762 M3 x 6:12
- Insert:6: XY_Plate:1 ↔ ISO 4762 M3 x 6:35
- Insert:7: XY_Plate:1 ↔ ISO 4762 M3 x 6:36
- Insert:8: XY_Plate:1 ↔ ISO 4762 M3 x 6:33
- Insert:9: XY_Plate:1 ↔ ISO 4762 M3 x 6:34
- Mate:149: Idler Left:1 ↔ V-Slot 20 x 20 20-20-V-slot 20 mm x 20 mm-Aluminum 6061-550:3
- Mate:150: Idler Left:1 ↔ V-Slot 20 x 20 20-20-V-slot 20 mm x 20 mm-Aluminum 6061-470:5
- Flush:85: Idler Left:1 ↔ V-Slot 20 x 20 20-20-V-slot 20 mm x 20 mm-Aluminum 6061-470:5
- Mate:151: XY_Carriage:1 ↔ MGN9C Block:2
- Mate:152: XY_Carriage:1 ↔ MGN9C Block:2
- Mate:153: XY_Carriage:1 ↔ MGN9C Block:2
- Mate:154: XY_Carriage:1 ↔ XY_Tensioner:1
- Mate:155: XY_Carriage:1 ↔ XY_Tensioner:1
- Mate:156 (2 mm): XY_Carriage:1 ↔ XY_Tensioner:1
- Mate:157: XY_Carriage:1 ↔ XY_Tensioner:2
- Mate:158: XY_Carriage:1 ↔ XY_Tensioner:2
- Mate:159 (2 mm): XY_Carriage:1 ↔ XY_Tensioner:2
- Mate:160: XY_Carriage:1 ↔ XY_Metal_Slug:1
- Mate:161: XY_Carriage:1 ↔ XY_Metal_Slug:1
- Mate:162: XY_Carriage:1 ↔ M3 Conical Washer:3
- Mate:163: XY_Carriage:1 ↔ M3 Conical Washer:1
- Mate:164: XY_Carriage:1 ↔ M3 Conical Washer:2
- Mate:165: XY_Carriage:1 ↔ M3 Conical Washer:4
- Mate:166: XY_Carriage:1 ↔ M3 Conical Washer:4
- Mate:167: XY_Carriage:1 ↔ M3 Conical Washer:3
- Mate:168: XY_Carriage:1 ↔ M3 Conical Washer:2
- Mate:169: XY_Carriage:1 ↔ M3 Conical Washer:1
- Mate:170: 6mm XY Packer Block:1 ↔ MGN9C Block:1
- Flush:86: 6mm XY Packer Block:1 ↔ MGN9C Block:1
- Flush:87: 6mm XY Packer Block:1 ↔ MGN9C Block:1
- Mate:171: 6mm XY Packer Block:2 ↔ MGN9C Block_MIR:1
- Flush:88: 6mm XY Packer Block:2 ↔ MGN9C Block_MIR:1
- Flush:89: 6mm XY Packer Block:2 ↔ MGN9C Block_MIR:1
- Mate:172: XY_Plate:1 ↔ 6mm XY Packer Block:2
## Named parameters: d13_d2 = 0 mm, d14_d3 = 0 mm, d15_d4 = -100 mm, d16_d5 = 0 mm, d17_d6 = 0 mm, d18_d7 = 0 mm, d19_d8 = 0 mm, d20_d9 = 0 mm, d21_d10 = 0 mm, d22_d0 = 0 mm, d23_d1 = 100 mm
